# Autodesk Inventor assembly: FinalFrameAssembly
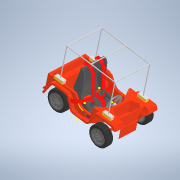
[picture p0: Inventor's stored thumbnail of the model, 180x180]
Saved by Autodesk Inventor 2021 (Build 250183000, 183)
## iProperties
Created: 2020-07-11
Part Number: FinalFrameAssembly
Document SubType Name: Assembly
Designer: Shannon
Author: Shannon
## Documents named in this file (7)
- C:\Users\Shannon\Documents\Non-MMAE Classes\IPRO S2020\FinalFrameAssembly.iam
- C:\Users\Shannon\Documents\Non-MMAE Classes\IPRO S2020\Jeep assembly.iam
- C:\Users\Shannon\Documents\Non-MMAE Classes\IPRO S2020\vertical support and 3 elbow.iam
- C:\Users\Shannon\Documents\Non-MMAE Classes\IPRO S2020\2ndvertical support and 3 elbow.iam
- C:\Users\Shannon\Documents\Non-MMAE Classes\IPRO S2020\horizontal support.ipt
- C:\Users\Shannon\Documents\Non-MMAE Classes\IPRO S2020\perpendicular horizontal bar.ipt
- C:\Users\Shannon\Documents\Non-MMAE Classes\IPRO S2020\bar elbow.ipt
## Components (12 placed, 6 different names)
1. Jeep assembly:1 [sub-assembly] — Mate:4, Mate:5, Mate:6, Mate:7, Mate:8, Mate:9, Mate:10, Mate:11, Mate:12, Mate:15, Mate:16, Mate:17
2. vertical support and 3 elbow:1 [sub-assembly] — Mate:4, Mate:5, Mate:6, Mate:14, Mate:21
3. vertical support and 3 elbow:2 [sub-assembly] — Mate:7, Mate:8, Mate:9, Mate:19, Mate:22
4. 2ndvertical support and 3 elbow:1 [sub-assembly] — Mate:10, Mate:11, Mate:12, Mate:18, Mate:20
5. horizontal support:1 — Mate:18, Mate:19, Mate:24, Mate:25
6. horizontal support:2 — Mate:14, Mate:28, Mate:29
7. 2ndvertical support and 3 elbow:2 [sub-assembly] — Mate:15, Mate:16, Mate:17, Mate:23, Mate:28
8. perpendicular horizontal bar:1 — Mate:22, Mate:23
9. perpendicular horizontal bar:3 — Mate:20, Mate:21
10. bar elbow:1 — Mate:24, Mate:25, Mate:30, Mate:32
11. bar elbow:2 — Mate:29, Mate:30, Mate:31
12. perpendicular horizontal bar:4 — Mate:31, Mate:32
## Relationships (26: Mate 26)
- Mate:4: Jeep assembly:1 ↔ vertical support and 3 elbow:1
- Mate:5: Jeep assembly:1 ↔ vertical support and 3 elbow:1
- Mate:6: Jeep assembly:1 ↔ vertical support and 3 elbow:1
- Mate:7: Jeep assembly:1 ↔ vertical support and 3 elbow:2
- Mate:8: Jeep assembly:1 ↔ vertical support and 3 elbow:2
- Mate:9: Jeep assembly:1 ↔ vertical support and 3 elbow:2
- Mate:10: Jeep assembly:1 ↔ 2ndvertical support and 3 elbow:1
- Mate:11: Jeep assembly:1 ↔ 2ndvertical support and 3 elbow:1
- Mate:12: Jeep assembly:1 ↔ 2ndvertical support and 3 elbow:1
- Mate:14: vertical support and 3 elbow:1 ↔ horizontal support:2
- Mate:15: Jeep assembly:1 ↔ 2ndvertical support and 3 elbow:2
- Mate:16: Jeep assembly:1 ↔ 2ndvertical support and 3 elbow:2
- Mate:17: Jeep assembly:1 ↔ 2ndvertical support and 3 elbow:2
- Mate:18: 2ndvertical support and 3 elbow:1 ↔ horizontal support:1
- Mate:19: vertical support and 3 elbow:2 ↔ horizontal support:1
- Mate:20: 2ndvertical support and 3 elbow:1 ↔ perpendicular horizontal bar:3
- Mate:21: vertical support and 3 elbow:1 ↔ perpendicular horizontal bar:3
- Mate:22: vertical support and 3 elbow:2 ↔ perpendicular horizontal bar:1
- Mate:23: 2ndvertical support and 3 elbow:2 ↔ perpendicular horizontal bar:1
- Mate:24: horizontal support:1 ↔ bar elbow:1
- Mate:25: horizontal support:1 ↔ bar elbow:1
- Mate:28: horizontal support:2 ↔ 2ndvertical support and 3 elbow:2
- Mate:29: horizontal support:2 ↔ bar elbow:2
- Mate:30: bar elbow:1 ↔ bar elbow:2
- Mate:31: bar elbow:2 ↔ perpendicular horizontal bar:4
- Mate:32: bar elbow:1 ↔ perpendicular horizontal bar:4
